# Autodesk Inventor assembly: 554211 ADNGF-12-40-P-A---(0)
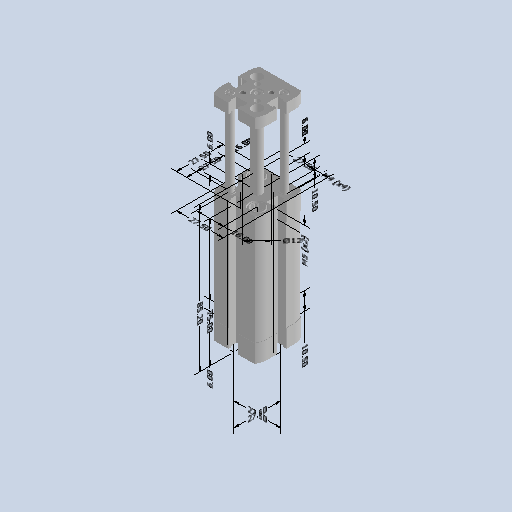
[picture p0: Inventor's stored thumbnail of the model, 512x512]
Saved by Autodesk Inventor 2025.2 (Build 292293000, 293)
## iProperties
Category: PARTsolutions
Company: FESTO
Created: 2025-06-05
Part Number: 554211 ADNGF-12-40-P-A---(0)
Catalog Web Link: www.cadenas.de
Description: ADNGF-Compact cylinder
Vendor: FESTO
Document SubType Name: Assembly
Designer: psAdmin
Manufacturer: FESTO
Mass: 132 g
Surface Area: 251.588 cm^2
Volume: 42.9819 cm^3
Density: 3.07106 g/cm^3
PSOL_IDENT_0: {ATYP=ASSISTANT},{DATA=script=$CADENAS_DATA/23d-libs/festo/webfesto.vbb&M_FAMILY=ADNGF&M_GROUP=01&M_
PSOL_IDENT_1: PARTNO=554211&IDCODE1=ADNGF-12-40-P-A&IDCODE2=&customer_number_cns=&MATES=1&LOD=HI&LOCKERP=0&SINGLEP
PSOL_IDENT_2: ART=1}
NB: 554211 ADNGF-12-40-P-A---(0)
NN: ADNGF
NT: Compact cylinder
NBSYN: $TNR. ADNGF-$KDM.-$HUB.-$DF.-$GA.---($HUBST.)
LINA: 554211 ADNGF-12-40-P-A
CATALOG: Festo
OFFICIAL_STANDARD_NUMBERS: ISO 21287
TNR: 554211
TYP: ADNGF-12-40-P-A
KDM: 12
HUB: 40
DF: P
GA: A
S2: -
HUBST: 0
AF: 8
BG: 17
D1: 9
D4: 12
D5: 6
D6: M3
D7: 0
E: 27.5
EE: M5
FB: 3
G: 10.5
J2: 2
J3: 0
KF: M3
LA: 3.5
ME: 6
MM: 6
PL: 6
RT: M4
SF: 5
T1: 0
T2: 2.1
T4: 1.5
TG: 16
WH: 4.2
ZA: 75
ZB: 39.2
ZM: 44.5
CNSMASSEXACT: 0.132
GTIN: 4052568198398
SUPPLIER: FESTO
ARTICLENO: 554211 ADNGF-12-40-P-A---(0)
BOMINFO: 554211 ADNGF-12-40-P-A
CREATOR: CADENAS GmbH
Title: 554211 ADNGF-12-40-P-A
Author: Cadenas PARTsolutions
Comments: Compact cylinder
## Documents named in this file (3)
- D:\Useless_Box\CAD-Paspa\Useless Box\Eigene Bauteile\JH_Greifer_Unterlegscheibe\Kaufteile\Führungszylinder\AIS2024\554211 ADNGF-12-40-P-A---(0).iam
- D:\Useless_Box\CAD-Paspa\Useless Box\Eigene Bauteile\JH_Greifer_Unterlegscheibe\Kaufteile\Führungszylinder\AIS2024\537123 ADNGF-12-40-P-A---(Z).ipt
- D:\Useless_Box\CAD-Paspa\Useless Box\Eigene Bauteile\JH_Greifer_Unterlegscheibe\Kaufteile\Führungszylinder\AIS2024\537123 ADNGF-12-40-P-A---(KS).ipt
## Components (2 placed, 2 different names)
1. 537123 ADNGF-12-40-P-A---(Z):1 — CYLINDER_XY@1 <-> PISTON_XY@2, CYLINDER_Z@1 <-> PISTON_Z@2, CYLINDER_YZ@1 <-> PISTON_YZ@2
2. 537123 ADNGF-12-40-P-A---(KS):1 — CYLINDER_XY@1 <-> PISTON_XY@2, CYLINDER_Z@1 <-> PISTON_Z@2, CYLINDER_YZ@1 <-> PISTON_YZ@2
## Relationships (3: Mate 2, Angle 1)
- CYLINDER_XY@1 <-> PISTON_XY@2 [Mate]: 537123 ADNGF-12-40-P-A---(Z):1 ↔ 537123 ADNGF-12-40-P-A---(KS):1
- CYLINDER_Z@1 <-> PISTON_Z@2 [Mate]: 537123 ADNGF-12-40-P-A---(Z):1 ↔ 537123 ADNGF-12-40-P-A---(KS):1
- CYLINDER_YZ@1 <-> PISTON_YZ@2 [Angle] (0 deg): 537123 ADNGF-12-40-P-A---(Z):1 ↔ 537123 ADNGF-12-40-P-A---(KS):1
